# Autodesk Inventor assembly: Main_Body_Assembly
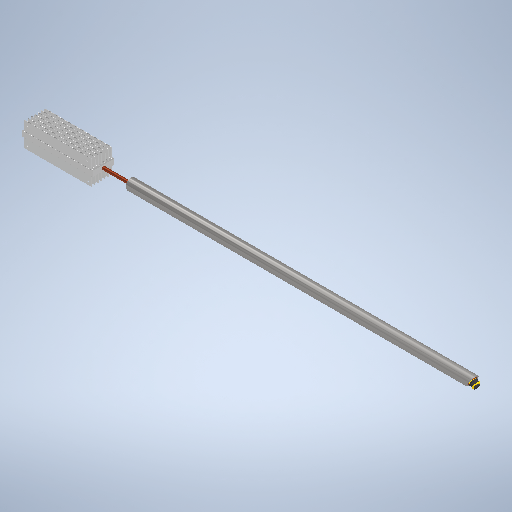
[picture p0: Inventor's stored thumbnail of the model, 512x512]
Saved by Autodesk Inventor 2026.2 (Build 302298010, 298A)
## iProperties
Created: 2026-05-12
Part Number: Main_Body_Assembly
Document SubType Name: Assembly
Designer: piete
Author: piete
## Documents named in this file (8)
- C:\Users\piete\Desktop\Skripsie\Documents\Detail Design\Main Body Design\Main_Body_Assembly.iam
- C:\Users\piete\Desktop\Skripsie\Documents\Detail Design\Main Body Design\Heat Sink Holed drilled.ipt
- C:\Users\piete\Desktop\Skripsie\Documents\Detail Design\Main Body Design\Heat Pipe 250 mm.ipt
- C:\Users\piete\Desktop\Skripsie\Documents\Detail Design\Main Body Design\Copper_Coupler.ipt
- C:\Users\piete\Desktop\Skripsie\Documents\Detail Design\Main Body Design\Heat Pipe 100 mm.ipt
- C:\Users\piete\Desktop\Skripsie\Documents\Detail Design\Main Body Design\Main_tip_coupler.ipt
- C:\Users\piete\Desktop\Skripsie\Documents\Detail Design\Main Body Design\Scaled Model.ipt
- C:\Users\piete\Desktop\Skripsie\Documents\Detail Design\Main Body Design\Stainless_Steel_Pipe.ipt
## Components (8 placed, 7 different names)
1. Heat Sink Holed drilled:1 — Flush:1, Mate:1, Flush:2, Mate:2, Mate:3
2. Heat Sink Holed drilled:2 — Flush:1, Mate:1, Flush:2, Flush:3
3. Heat Pipe 250 mm:1 — Mate:2, Mate:3, Flush:3, Mate:4, Mate:5, Mate:6
4. Copper_Coupler:1 — Mate:4, Mate:5, Mate:6, Mate:7, Mate:8, Mate:9
5. Heat Pipe 100 mm:1 — Mate:7, Mate:8, Mate:9, Mate:10, Mate:11, Mate:12, Mate:16
6. Main_tip_coupler:1 — Mate:10, Mate:11, Mate:12, Mate:13, Mate:14, Mate:15, Flush:4
7. Scaled Model:1 — Mate:13, Mate:14, Mate:15
8. Stainless_Steel_Pipe:1 — Flush:4, Mate:16
## Relationships (20: Mate 16, Flush 4)
- Flush:1: Heat Sink Holed drilled:1 ↔ Heat Sink Holed drilled:2
- Mate:1: Heat Sink Holed drilled:1 ↔ Heat Sink Holed drilled:2
- Flush:2: Heat Sink Holed drilled:1 ↔ Heat Sink Holed drilled:2
- Mate:2 (-30 mm): Heat Sink Holed drilled:1 ↔ Heat Pipe 250 mm:1
- Mate:3: Heat Sink Holed drilled:1 ↔ Heat Pipe 250 mm:1
- Flush:3: Heat Sink Holed drilled:2 ↔ Heat Pipe 250 mm:1
- Mate:4 (-18 mm): Heat Pipe 250 mm:1 ↔ Copper_Coupler:1
- Mate:5: Heat Pipe 250 mm:1 ↔ Copper_Coupler:1
- Mate:6: Heat Pipe 250 mm:1 ↔ Copper_Coupler:1
- Mate:7 (-12 mm): Copper_Coupler:1 ↔ Heat Pipe 100 mm:1
- Mate:8: Copper_Coupler:1 ↔ Heat Pipe 100 mm:1
- Mate:9: Copper_Coupler:1 ↔ Heat Pipe 100 mm:1
- Mate:10 (-13 mm): Heat Pipe 100 mm:1 ↔ Main_tip_coupler:1
- Mate:11: Heat Pipe 100 mm:1 ↔ Main_tip_coupler:1
- Mate:12: Heat Pipe 100 mm:1 ↔ Main_tip_coupler:1
- Mate:13 (0.2 mm): Main_tip_coupler:1 ↔ Scaled Model:1
- Mate:14: Main_tip_coupler:1 ↔ Scaled Model:1
- Mate:15: Main_tip_coupler:1 ↔ Scaled Model:1
- Flush:4: Main_tip_coupler:1 ↔ Stainless_Steel_Pipe:1
- Mate:16: Heat Pipe 100 mm:1 ↔ Stainless_Steel_Pipe:1
